# Autodesk Inventor assembly: Bottom Mold
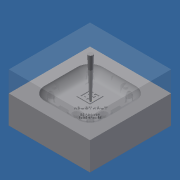
[picture p0: Inventor's stored thumbnail of the model, 180x180]
Saved by Autodesk Inventor 2016 (Build 200138000, 138)
## iProperties
Created: 2015-07-09
Part Number: Bottom Mold
Document SubType Name: Assembly
Designer: Samuel Clay
Author: Samuel Clay
## Documents named in this file (16)
- Z:\turntouch\remote\enclosure\inventor\Molds\Bottom Mold.iam
- Z:\turntouch\remote\enclosure\inventor\Molds\Bottom Mold_Remote Bottom_LY.iam
- Z:\turntouch\remote\enclosure\inventor\Molds\Bottom Mold_RG.ipt
- Z:\turntouch\remote\enclosure\inventor\Molds\AIT\Mold\MoldFlow\Bottom_20Mold_2Eiam\MITSI_Bottom_20Mold_2Eiam.mit
- Z:\turntouch\remote\enclosure\inventor\Molds\AIT\Mold\MoldFlow\Bottom_20Mold_2Eiam\bottom_20mold_5fremote_20bottom_5fmp_2eipt_gate.sdy
- Z:\turntouch\remote\enclosure\inventor\Molds\AIT\Mold\MoldFlow\Bottom_20Mold_2Eiam\bottom_20mold_5fremote_20bottom_5fmp_2eipt_gate~1.crc
- Z:\turntouch\remote\enclosure\inventor\Molds\AIT\Mold\MoldFlow\Bottom_20Mold_2Eiam\bottom_20mold_5fremote_20bottom_5fmp_2eipt_gate~1.ot1
- Z:\turntouch\remote\enclosure\inventor\Molds\AIT\Mold\MoldFlow\Bottom_20Mold_2Eiam\bottom_20mold_5fremote_20bottom_5fmp_2eipt_gate~1.out
- Z:\turntouch\remote\enclosure\inventor\Molds\AIT\Mold\MoldFlow\Bottom_20Mold_2Eiam\bottom_20mold_5fremote_20bottom_5fmp_2eipt_gate~1.rfn
- Z:\turntouch\remote\enclosure\inventor\Molds\AIT\Mold\MoldFlow\Bottom_20Mold_2Eiam\bottom_20mold_5fremote_20bottom_5fmp_2eipt_gate~2Check.rfn
- Z:\turntouch\remote\enclosure\inventor\Molds\AIT\Mold\MoldFlow\Bottom_20Mold_2Eiam\bottom_20mold_5fremote_20bottom_5fmp_2eipt_gate~3User.rfn
- Z:\turntouch\remote\enclosure\inventor\Molds\AIT\Mold\MoldFlow\Bottom_20Mold_2Eiam\bottom_20mold_5fremote_20bottom_5fmp_2eipt_gate~4Doe.rfn
- Z:\turntouch\remote\enclosure\inventor\Molds\AIT\Mold\MoldFlow\Bottom_20Mold_2Eiam\bottom_20mold_5fremote_20bottom_5fmp_2eipt_gate~5Mesh.crc
- Z:\turntouch\remote\enclosure\inventor\Molds\AIT\Mold\MoldFlow\Bottom_20Mold_2Eiam\bottom_20mold_5fremote_20bottom_5fmp_2eipt_gate~5Mesh.of1
- Z:\turntouch\remote\enclosure\inventor\Molds\AIT\Mold\MoldFlow\Bottom_20Mold_2Eiam\bottom_20mold_5fremote_20bottom_5fmp_2eipt_gate~5Mesh.out
- Z:\turntouch\remote\enclosure\inventor\Molds\AIT\Mold\MoldFlow\Bottom_20Mold_2Eiam\bottom_20mold_5fremote_20bottom_5fmp_2eipt_gate~5Mesh.rfn
## Components (2 placed, 2 different names)
1. Bottom Mold_Remote Bottom_LY:1 [sub-assembly] — Flush:1, Flush:2, Flush:3
2. Bottom Mold_RG:1
## Relationships (3: Flush 3)
- Flush:1: Bottom Mold_Remote Bottom_LY:1
- Flush:2: Bottom Mold_Remote Bottom_LY:1
- Flush:3: Bottom Mold_Remote Bottom_LY:1
